# Autodesk Inventor assembly: Assembly1
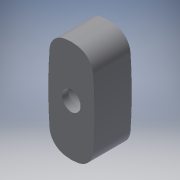
[picture p0: Inventor's stored thumbnail of the model, 180x180]
Saved by Autodesk Inventor 2017 (Build 210142000, 142)
## iProperties
Created: 2019-06-26
Part Number: Assembly1
Document SubType Name: Assembly
Designer: Ole Simmering
Author: Ole Simmering
## Documents named in this file (3)
- C:\Users\Ole Simmering\Documents\GitHub\3D_modeling\Kopfhörer Ersatzteil\Assembly1.iam
- C:\Users\Ole Simmering\Documents\GitHub\3D_modeling\Kopfhörer Ersatzteil\Part1.ipt
- C:\Users\Ole Simmering\Documents\GitHub\3D_modeling\Kopfhörer Ersatzteil\Part2.ipt
## Components (2 placed, 2 different names)
1. Part1:1 — Angle:1, Mate:1, Mate:2, Insert:1
2. Part2:1 — Angle:1, Mate:1, Mate:2, Insert:1
## Relationships (4: Mate 2, Angle 1, Insert 1)
- Angle:1 (0 deg): Part1:1 ↔ Part2:1
- Mate:1: Part1:1 ↔ Part2:1
- Mate:2: Part1:1 ↔ Part2:1
- Insert:1: Part1:1 ↔ Part2:1
